# Autodesk Inventor assembly: tower
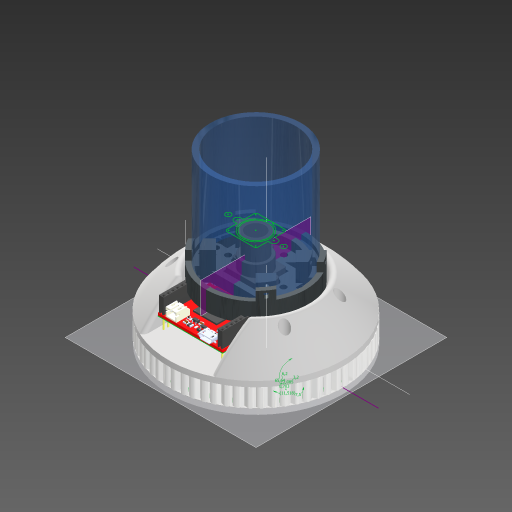
[picture p0: Inventor's stored thumbnail of the model, 512x512]
Saved by Autodesk Inventor 2023 (Build 270158000, 158)
## iProperties
Created: 2025-07-01
Part Number: tower
Document SubType Name: Assembly
Designer: daa
Author: daa
## Documents named in this file (5)
- C:\Users\daa\Documents\DASH_V2\tower.iam
- C:\Users\daa\Documents\DASH_V2\openmv_cennt.iam
- C:\Users\daa\Documents\DASH_V2\openmv.ipt
- C:\Users\daa\Documents\DASH_V2\openmv_cr.ipt
- C:\Users\daa\Documents\DASH_V2\tssop.iam
## Components (4 placed, 4 different names)
1. openmv_cennt:1 [sub-assembly] — С поворотом:1
2. openmv:1 — С поворотом:1, С поворотом:2, С поворотом:3
3. openmv_cr:1 — С поворотом:2
4. tssop:1 [sub-assembly] — С поворотом:3
## Relationships (3: RevoluteJoint 3)
- С поворотом:1 [RevoluteJoint]: openmv_cennt:1 ↔ openmv:1
- С поворотом:2 [RevoluteJoint]: openmv:1 ↔ openmv_cr:1
- С поворотом:3 [RevoluteJoint]: openmv:1 ↔ tssop:1
